# Autodesk Inventor assembly: Assembly1
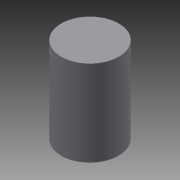
[picture p0: Inventor's stored thumbnail of the model, 180x180]
Saved by Autodesk Inventor 2015 (Build 190159000, 159)
## iProperties
Created: 2018-04-06
Part Number: Assembly1
Document SubType Name: Assembly
Designer: Administrator
Author: Administrator
## Documents named in this file (4)
- L:\IED 9th\Science Pop Can Lab\Assembly1.iam
- L:\IED 9th\Science Pop Can Lab\Inner Layer.ipt
- L:\IED 9th\Science Pop Can Lab\Outer Layer.ipt
- L:\IED 9th\Science Pop Can Lab\Lid.ipt
## Components (3 placed, 3 different names)
1. Inner Layer:1 — Insert:1
2. Outer Layer:1 — Insert:1, Mate:1
3. Lid:1 — Mate:1
## Relationships (2: Insert 1, Mate 1)
- Insert:1: Inner Layer:1 ↔ Outer Layer:1
- Mate:1: Outer Layer:1 ↔ Lid:1
